# Autodesk Inventor assembly: A2017_T2_01
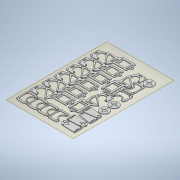
[picture p0: Inventor's stored thumbnail of the model, 180x180]
Saved by Autodesk Inventor 2020 (Build 240168000, 168)
## iProperties
Created: 2021-08-27
Part Number: A2017_T2_01
Document SubType Name: Assembly
Designer: Masato
Author: Masato
## Documents named in this file (7)
- C:\Users\naoki\Documents\Inventor\CitBrains\git_clone\SUSTAINA_ver1_0\治具\SUSTAINA-OP\Cam\A2017_T2_01.iam
- C:\Users\naoki\Documents\Inventor\CitBrains\git_clone\SUSTAINA_ver1_0\治具\SUSTAINA-OP\Cam\DisposableBoard.ipt
- C:\Users\naoki\Documents\Inventor\CitBrains\git_clone\SUSTAINA_ver1_0\治具\SUSTAINA-OP\LowerBody\Ankle\Ankle_back_frame.ipt
- C:\Users\naoki\Documents\Inventor\CitBrains\git_clone\SUSTAINA_ver1_0\治具\SUSTAINA-OP\LowerBody\Foot\Foot_back_frame.ipt
- C:\Users\naoki\Documents\Inventor\CitBrains\git_clone\SUSTAINA_ver1_0\治具\SUSTAINA-OP\LowerBody\Foot\Foot_front_frame.ipt
- C:\Users\naoki\Documents\Inventor\CitBrains\git_clone\SUSTAINA_ver1_0\治具\SUSTAINA-OP\LowerBody\Ankle\Ankle_side_frame.ipt
- C:\Users\naoki\Documents\Inventor\CitBrains\git_clone\SUSTAINA_ver1_0\治具\SUSTAINA-OP\UpperBody\Trunk\CrossRollerBearing\Inner_flange.ipt
## Components (22 placed, 6 different names)
1. DisposableBoard:1 — メイト:2, メイト:1, フラッシュ:1, フラッシュ:2, メイト:4, メイト:5, メイト:6, メイト:7, メイト:9, メイト:10, メイト:11, メイト:12, メイト:13, メイト:17, メイト:18, メイト:19, メイト:20, メイト:21, メイト:22, メイト:23, 正接:1, 正接:3, メイト:36, メイト:46, メイト:47, 角度:1, 角度:2, フラッシュ:3, メイト:50, 正接:11, 正接:12, メイト:54, メイト:55, メイト:56, 角度:3
2. Ankle_back_frame:1 — メイト:4, メイト:9, メイト:10, メイト:14, メイト:48
3. Ankle_back_frame:2 — メイト:5, メイト:11, メイト:14, メイト:15
4. Ankle_back_frame:3 — メイト:6, メイト:12, メイト:15, メイト:16
5. Ankle_back_frame:4 — メイト:7, メイト:13, メイト:16
6. Foot_back_frame:2 — メイト:19, メイト:22, メイト:23, メイト:24
7. Foot_front_frame:1 — メイト:17, メイト:21, 正接:2, メイト:25
8. Foot_front_frame:2 — メイト:18, メイト:25, 正接:3, 正接:9, 正接:13
9. Foot_back_frame:3 — メイト:20, 正接:1, メイト:24, 正接:2
10. Inner_flange:1 — メイト:46, 角度:1, 正接:9, 正接:10, 正接:11
11. Inner_flange:2 — メイト:47, 正接:10, 角度:2, 正接:12
12. Ankle_back_frame:5 — メイト:53, 正接:14, 正接:15, メイト:55
13. Ankle_back_frame:6 — メイト:51, メイト:52, メイト:53, メイト:56
14. Inner_flange:3 — 正接:15, 正接:16, メイト:54, 角度:3
15. Ankle_side_frame:1 — メイト:36, メイト:48, フラッシュ:3, メイト:49
16. Ankle_side_frame:2
17. Ankle_side_frame:3
18. Ankle_side_frame:5
19. Ankle_side_frame:6
20. Ankle_side_frame:7
21. Ankle_side_frame:4 — メイト:49, メイト:50, 正接:13, メイト:51
22. Ankle_side_frame:9 — メイト:52, 正接:14, 正接:16
## Component patterns: (6 elements, first: Ankle_side_frame:1), (2 elements, first: Ankle_side_frame:4)
## Relationships (52: Mate 35, Tangent 11, Flush 3, Angle 3)
- メイト:2 [Mate]: DisposableBoard:1
- メイト:1 [Mate]: DisposableBoard:1
- フラッシュ:1 [Flush]: DisposableBoard:1
- フラッシュ:2 [Flush]: DisposableBoard:1
- メイト:4 [Mate]: DisposableBoard:1 ↔ Ankle_back_frame:1
- メイト:5 [Mate]: DisposableBoard:1 ↔ Ankle_back_frame:2
- メイト:6 [Mate]: DisposableBoard:1 ↔ Ankle_back_frame:3
- メイト:7 [Mate]: DisposableBoard:1 ↔ Ankle_back_frame:4
- メイト:9 [Mate] (3 mm): DisposableBoard:1 ↔ Ankle_back_frame:1
- メイト:10 [Mate] (3 mm): DisposableBoard:1 ↔ Ankle_back_frame:1
- メイト:11 [Mate] (3 mm): DisposableBoard:1 ↔ Ankle_back_frame:2
- メイト:12 [Mate] (3 mm): DisposableBoard:1 ↔ Ankle_back_frame:3
- メイト:13 [Mate] (3 mm): DisposableBoard:1 ↔ Ankle_back_frame:4
- メイト:14 [Mate] (2.5 mm): Ankle_back_frame:1 ↔ Ankle_back_frame:2
- メイト:15 [Mate] (2.5 mm): Ankle_back_frame:2 ↔ Ankle_back_frame:3
- メイト:16 [Mate] (2.5 mm): Ankle_back_frame:3 ↔ Ankle_back_frame:4
- メイト:17 [Mate]: DisposableBoard:1 ↔ Foot_front_frame:1
- メイト:18 [Mate]: DisposableBoard:1 ↔ Foot_front_frame:2
- メイト:19 [Mate]: DisposableBoard:1 ↔ Foot_back_frame:2
- メイト:20 [Mate]: DisposableBoard:1 ↔ Foot_back_frame:3
- メイト:21 [Mate] (3 mm): DisposableBoard:1 ↔ Foot_front_frame:1
- メイト:22 [Mate] (3 mm): DisposableBoard:1 ↔ Foot_back_frame:2
- メイト:23 [Mate] (3 mm): DisposableBoard:1 ↔ Foot_back_frame:2
- 正接:1 [Tangent] (3 mm): DisposableBoard:1 ↔ Foot_back_frame:3
- メイト:24 [Mate] (2.5 mm): Foot_back_frame:2 ↔ Foot_back_frame:3
- 正接:2 [Tangent] (2.5 mm): Foot_front_frame:1 ↔ Foot_back_frame:3
- メイト:25 [Mate] (2.5 mm): Foot_front_frame:1 ↔ Foot_front_frame:2
- 正接:3 [Tangent] (3 mm): DisposableBoard:1 ↔ Foot_front_frame:2
- メイト:36 [Mate]: DisposableBoard:1 ↔ Ankle_side_frame:1
- メイト:46 [Mate]: DisposableBoard:1 ↔ Inner_flange:1
- メイト:47 [Mate]: DisposableBoard:1 ↔ Inner_flange:2
- 角度:1 [Angle] (0 deg): DisposableBoard:1 ↔ Inner_flange:1
- 正接:9 [Tangent] (2.5 mm): Foot_front_frame:2 ↔ Inner_flange:1
- 正接:10 [Tangent] (2.5 mm): Inner_flange:1 ↔ Inner_flange:2
- 角度:2 [Angle] (0 deg): DisposableBoard:1 ↔ Inner_flange:2
- メイト:48 [Mate] (2.5 mm): Ankle_back_frame:1 ↔ Ankle_side_frame:1
- フラッシュ:3 [Flush] (2 mm): DisposableBoard:1 ↔ Ankle_side_frame:1
- メイト:49 [Mate] (2.5 mm): Ankle_side_frame:1 ↔ Ankle_side_frame:4
- メイト:50 [Mate]: DisposableBoard:1 ↔ Ankle_side_frame:4
- 正接:11 [Tangent] (2.5 mm): DisposableBoard:1 ↔ Inner_flange:1
- 正接:12 [Tangent] (2.5 mm): DisposableBoard:1 ↔ Inner_flange:2
- 正接:13 [Tangent] (2.5 mm): Foot_front_frame:2 ↔ Ankle_side_frame:4
- メイト:51 [Mate] (2.5 mm): Ankle_back_frame:6 ↔ Ankle_side_frame:4
- メイト:52 [Mate] (2.5 mm): Ankle_back_frame:6 ↔ Ankle_side_frame:9
- メイト:53 [Mate] (2.5 mm): Ankle_back_frame:5 ↔ Ankle_back_frame:6
- 正接:14 [Tangent] (2.5 mm): Ankle_back_frame:5 ↔ Ankle_side_frame:9
- 正接:15 [Tangent] (2.5 mm): Ankle_back_frame:5 ↔ Inner_flange:3
- 正接:16 [Tangent] (2.5 mm): Inner_flange:3 ↔ Ankle_side_frame:9
- メイト:54 [Mate]: DisposableBoard:1 ↔ Inner_flange:3
- メイト:55 [Mate]: DisposableBoard:1 ↔ Ankle_back_frame:5
- メイト:56 [Mate]: DisposableBoard:1 ↔ Ankle_back_frame:6
- 角度:3 [Angle] (0 deg): DisposableBoard:1 ↔ Inner_flange:3
